# Autodesk Inventor assembly: longarms
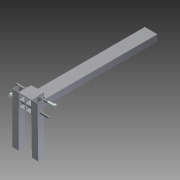
[picture p0: Inventor's stored thumbnail of the model, 180x180]
Saved by Autodesk Inventor 2011 (Build 150239000, 239)
## iProperties
Created: 2013-01-19
Part Number: longarms
Document SubType Name: Assembly
Designer: Danny
Author: Danny
## Documents named in this file (6)
- C:\Users\Danny\Documents\GitHub\2013CAD\2013 robot\Spiderbot\longarms.iam
- C:\Users\Danny\Documents\GitHub\2013CAD\2013 robot\Spiderbot\var in 1-16.ipt
- C:\Users\Danny\Documents\GitHub\2013CAD\2013 robot\Spiderbot\2 in 1-16.ipt
- C:\Users\Danny\Documents\GitHub\2013CAD\2013 robot\Spiderbot\long hex bolt.ipt
- C:\Users\Danny\Documents\GitHub\2013CAD\2013 robot\Spiderbot\nylock nut.ipt
- C:\Users\Danny\Documents\GitHub\2013CAD\2013 robot\Spiderbot\8 in 1-16.ipt
## Components (10 placed, 5 different names)
1. var in 1-16:1 — Mate:1, Flush:1, Flush:2, Mate:2, Flush:3, Flush:6, Mate:4, Mate:11
2. var in 1-16:2 — Mate:1, Flush:1, Flush:2, Mate:3, Flush:5, Mate:14
3. 2 in 1-16:1 — Mate:2, Flush:3, Flush:4, Flush:6, Mate:12
4. 2 in 1-16:2 — Mate:3, Flush:4, Flush:5, Mate:18
5. Chassis_HexBolt_375x16x7_AndyMark_am-1055:1 — Mate:4, Mate:10, Mate:13
6. 8 in 1-16:1 — Mate:13, Mate:14
7. 8 in 1-16:2 — Mate:10, Mate:11
8. Chassis_HexBolt_375x16x7_AndyMark_am-1055:2 — Mate:12, Mate:15, Mate:16, Mate:17
9. nylock nut:1 — Mate:15
10. nylock nut:2 — Mate:16, Mate:17, Mate:18
## Relationships (19: Mate 13, Flush 6)
- Mate:1: var in 1-16:1 ↔ var in 1-16:2
- Flush:1: var in 1-16:1 ↔ var in 1-16:2
- Flush:2: var in 1-16:1 ↔ var in 1-16:2
- Mate:2: var in 1-16:1 ↔ 2 in 1-16:1
- Flush:3: var in 1-16:1 ↔ 2 in 1-16:1
- Mate:3: var in 1-16:2 ↔ 2 in 1-16:2
- Flush:4: 2 in 1-16:1 ↔ 2 in 1-16:2
- Flush:5: var in 1-16:2 ↔ 2 in 1-16:2
- Flush:6: var in 1-16:1 ↔ 2 in 1-16:1
- Mate:4: var in 1-16:1 ↔ Chassis_HexBolt_375x16x7_AndyMark_am-1055:1
- Mate:10: Chassis_HexBolt_375x16x7_AndyMark_am-1055:1 ↔ 8 in 1-16:2
- Mate:11: var in 1-16:1 ↔ 8 in 1-16:2
- Mate:12: 2 in 1-16:1 ↔ Chassis_HexBolt_375x16x7_AndyMark_am-1055:2
- Mate:13: Chassis_HexBolt_375x16x7_AndyMark_am-1055:1 ↔ 8 in 1-16:1
- Mate:14: var in 1-16:2 ↔ 8 in 1-16:1
- Mate:15: Chassis_HexBolt_375x16x7_AndyMark_am-1055:2 ↔ nylock nut:1
- Mate:16: Chassis_HexBolt_375x16x7_AndyMark_am-1055:2 ↔ nylock nut:2
- Mate:17: Chassis_HexBolt_375x16x7_AndyMark_am-1055:2 ↔ nylock nut:2
- Mate:18: 2 in 1-16:2 ↔ nylock nut:2
